# Autodesk Inventor assembly: FullSkirt
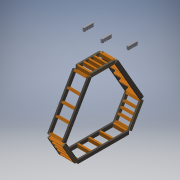
[picture p0: Inventor's stored thumbnail of the model, 180x180]
Saved by Autodesk Inventor 2016 (Build 200138000, 138)
## iProperties
Created: 2016-06-15
Part Number: FullSkirt
Document SubType Name: Assembly
Designer: cutrones
Author: cutrones
## Documents named in this file (4)
- C:\Users\cutrones\Desktop\MotionBase\CAD\MotionBaseCAD\BaseSkirt\FullSkirt.iam
- C:\Users\cutrones\Desktop\MotionBase\CAD\MotionBaseCAD\BaseSkirt\LargeSkirtWall.iam
- C:\Users\cutrones\Desktop\MotionBase\CAD\MotionBaseCAD\BaseSkirt\SmallSkirtWall.iam
- C:\Users\cutrones\Desktop\MotionBase\CAD\MotionBaseCAD\BaseSkirt\LargeSideHook.ipt
## Components (9 placed, 3 different names)
1. LargeSkirtWall:1 [sub-assembly] — Mate:5, Flush:4, Flush:5, Mate:7, Angle:2, Mate:8, Mate:9
2. LargeSkirtWall:2 [sub-assembly] — Mate:2, Mate:3, Flush:3, Flush:6, Angle:1
3. LargeSkirtWall:3 [sub-assembly] — Mate:1, Mate:6, Flush:1, Flush:2, Angle:3
4. SmallSkirtWall:1 [sub-assembly] — Mate:3, Flush:5, Flush:6, Mate:7, Angle:3
5. SmallSkirtWall:2 [sub-assembly] — Mate:5, Mate:6, Flush:1, Flush:4, Angle:1
6. SmallSkirtWall:3 [sub-assembly] — Mate:1, Mate:2, Flush:2, Flush:3, Angle:2
7. LargeSideHook:1
8. LargeSideHook:2
9. LargeSideHook:3
## Relationships (17: Mate 8, Flush 6, Angle 3)
- Mate:1: LargeSkirtWall:3 ↔ SmallSkirtWall:3
- Mate:2: LargeSkirtWall:2 ↔ SmallSkirtWall:3
- Mate:3: LargeSkirtWall:2 ↔ SmallSkirtWall:1
- Mate:5: LargeSkirtWall:1 ↔ SmallSkirtWall:2
- Mate:6: LargeSkirtWall:3 ↔ SmallSkirtWall:2
- Flush:1: LargeSkirtWall:3 ↔ SmallSkirtWall:2
- Flush:2: LargeSkirtWall:3 ↔ SmallSkirtWall:3
- Flush:3: LargeSkirtWall:2 ↔ SmallSkirtWall:3
- Flush:4: LargeSkirtWall:1 ↔ SmallSkirtWall:2
- Flush:5: LargeSkirtWall:1 ↔ SmallSkirtWall:1
- Flush:6: LargeSkirtWall:2 ↔ SmallSkirtWall:1
- Mate:7: LargeSkirtWall:1 ↔ SmallSkirtWall:1
- Angle:1 (0 deg): LargeSkirtWall:2 ↔ SmallSkirtWall:2
- Angle:2 (180 deg): LargeSkirtWall:1 ↔ SmallSkirtWall:3
- Angle:3 (180 deg): LargeSkirtWall:3 ↔ SmallSkirtWall:1
- Mate:8: LargeSkirtWall:1
- Mate:9: LargeSkirtWall:1
